# Autodesk Inventor assembly: poleAssembly
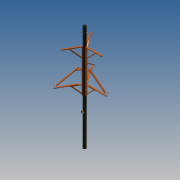
[picture p0: Inventor's stored thumbnail of the model, 180x180]
Saved by Autodesk Inventor 2014 SP1 (Build 180222100, 222)
## iProperties
Created: 2014-08-25
Part Number: poleAssembly
Document SubType Name: Assembly
Designer: Dave
Author: Dave
## Documents named in this file (10)
- C:\Users\Dave\Desktop\hera-cad\support\poleAssembly.iam
- C:\Users\Dave\Desktop\hera-cad\support\pole.ipt
- C:\Users\Dave\Desktop\hera-cad\support\heightMarker.ipt
- C:\Users\Dave\Desktop\hera-cad\support\poleStandVertAssy.iam
- C:\Users\Dave\Desktop\hera-cad\support\poleStandHorizAssy.iam
- C:\Users\Dave\Desktop\hera-cad\smallParts\eyebolt_ss_375.ipt
- C:\Users\Dave\Desktop\hera-cad\smallParts\pulley.ipt
- C:\Users\Dave\Desktop\hera-cad\support\winchAssembly.iam
- C:\Users\Dave\Desktop\hera-cad\smallParts\eyebolt_small.ipt
- C:\Users\Dave\Desktop\hera-cad\support\feedCableStay.iam
## Components (21 placed, 9 different names)
1. pole:1 — Insert:1, Mate:4, Flush:2, Insert:2, Insert:3, Mate:5
2. heightMarker:1 — Insert:1, Mate:1
3. winchAssembly:1 [sub-assembly]
4. poleStandVertAssy:1 [sub-assembly] — Mate:1, Mate:2, Flush:1, Mate:3, Mate:4, Flush:2, Flush:3
5. poleStandHorizAssy:1 [sub-assembly] — Mate:2, Flush:1, Mate:3
6. eyebolt_ss_375:1 — Insert:2
7. pulley:1
8. eyebolt_small:1 — Insert:3
9. feedCableStay:1 [sub-assembly] — Mate:5, Flush:3
10. poleStandVertAssy:2 [sub-assembly]
11. poleStandHorizAssy:2 [sub-assembly]
12. eyebolt_ss_375:2
13. pulley:2
14. eyebolt_small:2
15. feedCableStay:2 [sub-assembly]
16. poleStandVertAssy:3 [sub-assembly]
17. poleStandHorizAssy:3 [sub-assembly]
18. eyebolt_ss_375:3
19. pulley:3
20. eyebolt_small:3
21. feedCableStay:3 [sub-assembly]
## Component patterns: supports (3 elements)
## Relationships (11: Mate 5, Insert 3, Flush 3)
- Insert:1 (-2143.76 mm): pole:1 ↔ heightMarker:1
- Mate:1 (924.56 mm): heightMarker:1 ↔ poleStandVertAssy:1
- Mate:2: poleStandVertAssy:1 ↔ poleStandHorizAssy:1
- Flush:1: poleStandVertAssy:1 ↔ poleStandHorizAssy:1
- Mate:3 (162.56 mm): poleStandVertAssy:1 ↔ poleStandHorizAssy:1
- Mate:4: pole:1 ↔ poleStandVertAssy:1
- Flush:2 (57.15 mm): pole:1 ↔ poleStandVertAssy:1
- Insert:2 (-50.8 mm): pole:1 ↔ eyebolt_ss_375:1
- Insert:3 (-7.62 mm): pole:1 ↔ eyebolt_small:1
- Mate:5: pole:1 ↔ feedCableStay:1
- Flush:3 (304.8 mm): poleStandVertAssy:1 ↔ feedCableStay:1
